# Autodesk Inventor assembly: Bumper
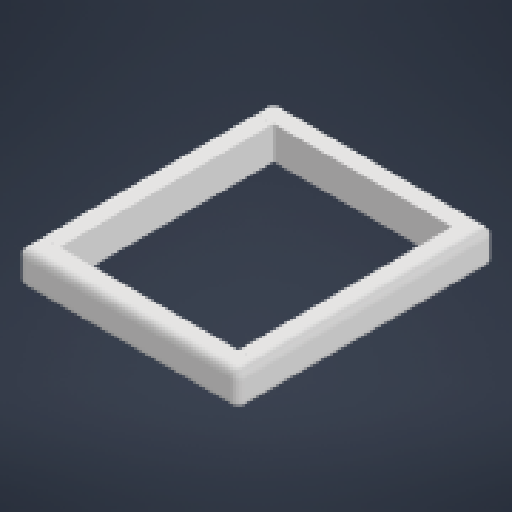
[picture p0: Inventor's stored thumbnail of the model, 512x512]
Saved by Autodesk Inventor 2023 (Build 270158000, 158)
## iProperties
Created: 2023-01-12
Part Number: Bumper
Document SubType Name: Assembly
Designer: Blank Slate
Author: Blank Slate
## Documents named in this file (3)
- C:\Users\Blank Slate\Documents\FRC 2023\Bumper.iam
- C:\Users\Blank Slate\Documents\FRC 2023\Solid2.ipt
- C:\Users\Blank Slate\Documents\FRC 2023\Solid1_2.ipt
## Components (4 placed, 2 different names)
1. Solid2:1 — Flush:3, Flush:4
2. Solid1_2:1 — Mate:2
3. Solid2:2 — Mate:1, Flush:1, Flush:2, Mate:2
4. Solid1_2:2 — Mate:1, Flush:1, Flush:2, Flush:3, Flush:4
## Relationships (6: Flush 4, Mate 2)
- Mate:1: Solid2:2 ↔ Solid1_2:2
- Flush:1: Solid2:2 ↔ Solid1_2:2
- Flush:2: Solid2:2 ↔ Solid1_2:2
- Mate:2: Solid1_2:1 ↔ Solid2:2
- Flush:3: Solid2:1 ↔ Solid1_2:2
- Flush:4: Solid2:1 ↔ Solid1_2:2
